# Autodesk Inventor assembly: ParticleLauncherwCollector
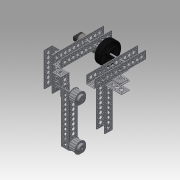
[picture p0: Inventor's stored thumbnail of the model, 180x180]
Saved by Autodesk Inventor 2016 (Build 200138000, 138)
## iProperties
Created: 2016-10-12
Part Number: ParticleLauncherwCollector
Document SubType Name: Assembly
Designer: Delta
Author: Delta
## Documents named in this file (12)
- C:\Robotics\2016-17_CAD\ParticleLauncherwCollector.iam
- C:\Robotics\CAD\2015-16\COTSParts\Actobotics\585 parts\585450.ipt
- C:\Robotics\CAD\2015-16\COTSParts\Actobotics\585 parts\585446.ipt
- C:\Robotics\CAD\2015-16\COTSParts\Actobotics\585 parts\585484.ipt
- C:\Robotics\CAD\2015-16\COTSParts\Actobotics\585 parts\585440.ipt
- C:\Robotics\CAD\2015-16\COTSParts\Actobotics\555 parts\555116.ipt
- C:\Robotics\CAD\2015-16\COTSParts\Actobotics\am-3102NeveRest20 (1).ipt
- C:\Robotics\CAD\2015-16\COTSParts\Actobotics\634 parts\634088.ipt
- C:\Users\Delta\Downloads\4in Wheel Intergreated Hub 8mm Rev2.ipt
- C:\Robotics\CAD\2015-16\COTSParts\Brecoflex\ls40t10_15-2_hub-32x10_d-8h7.ipt
- C:\Robotics\CAD\2015-16\COTSParts\Actobotics\634 parts\634080.ipt
- C:\Robotics\CAD\2015-16\COTSParts\Actobotics\634 parts\634078.ipt
## Components (17 placed, 11 different names)
1. 585450:1 — Mate:1, Flush:1, Flush:4, Insert:11, Insert:12
2. 585450:2 — Mate:1, Flush:1, Mate:2, Flush:2, Flush:3, Flush:4, Insert:13, Insert:14, Insert:16
3. 585446:1 — Mate:2, Flush:2, Flush:3, Insert:1, Insert:2
4. 585484:1 — Insert:1, Insert:2, Insert:3, Insert:4, Insert:21
5. 585450:3 — Insert:3, Insert:4, Insert:19, Insert:20, Insert:22
6. 585440:1 — Insert:7, Insert:8, Insert:11, Insert:12
7. 585484:2 — Insert:7, Insert:8, Insert:9, Insert:10
8. 585450:4 — Insert:9, Insert:10
9. 555116:1 — Insert:13, Insert:14, Insert:15
10. am-3102NeveRest20 (1):1 — Insert:15, Insert:18
11. 634088:1 — Insert:16, Insert:17
12. 4in Wheel Intergreated Hub 8mm Rev2:1 — Insert:17
13. 4in Wheel Intergreated Hub 8mm Rev2:2 — Insert:18
14. ls40t10_15-2_hub-32x10_d-8h7:1 — Insert:19
15. ls40t10_15-2_hub-32x10_d-8h7:2 — Insert:20
16. 634080:1 — Insert:21
17. 634078:1 — Insert:22
## Relationships (26: Insert 20, Flush 4, Mate 2)
- Mate:1 (114.3 mm): 585450:1 ↔ 585450:2
- Flush:1: 585450:1 ↔ 585450:2
- Mate:2: 585450:2 ↔ 585446:1
- Flush:2: 585450:2 ↔ 585446:1
- Flush:3: 585450:2 ↔ 585446:1
- Insert:1: 585446:1 ↔ 585484:1
- Insert:2: 585446:1 ↔ 585484:1
- Flush:4: 585450:1 ↔ 585450:2
- Insert:3: 585484:1 ↔ 585450:3
- Insert:4: 585484:1 ↔ 585450:3
- Insert:7: 585440:1 ↔ 585484:2
- Insert:8: 585440:1 ↔ 585484:2
- Insert:9: 585484:2 ↔ 585450:4
- Insert:10: 585484:2 ↔ 585450:4
- Insert:11: 585450:1 ↔ 585440:1
- Insert:12: 585450:1 ↔ 585440:1
- Insert:13: 585450:2 ↔ 555116:1
- Insert:14: 585450:2 ↔ 555116:1
- Insert:15 (-9.525 mm): 555116:1 ↔ am-3102NeveRest20 (1):1
- Insert:16 (19.05 mm): 585450:2 ↔ 634088:1
- Insert:17 (76.2 mm): 634088:1 ↔ 4in Wheel Intergreated Hub 8mm Rev2:1
- Insert:18 (-19.05 mm): am-3102NeveRest20 (1):1 ↔ 4in Wheel Intergreated Hub 8mm Rev2:2
- Insert:19: 585450:3 ↔ ls40t10_15-2_hub-32x10_d-8h7:1
- Insert:20: 585450:3 ↔ ls40t10_15-2_hub-32x10_d-8h7:2
- Insert:21 (-22.225 mm): 585484:1 ↔ 634080:1
- Insert:22 (-6.35 mm): 585450:3 ↔ 634078:1
